# Autodesk Inventor assembly: ASY PNS 1650 filter-distribution-system 1000
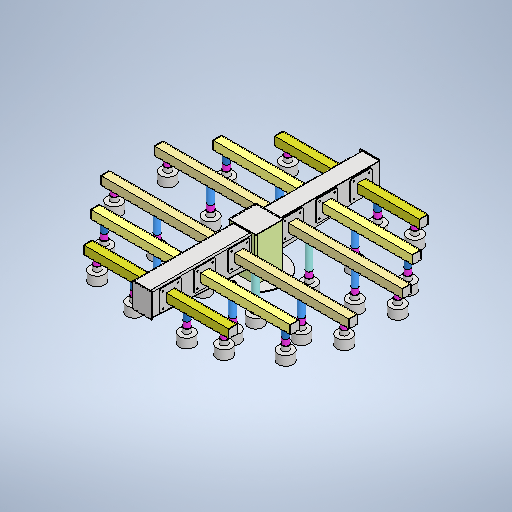
[picture p0: Inventor's stored thumbnail of the model, 512x512]
Saved by Autodesk Inventor 2025.3 (Build 293356030, 356C)
## iProperties
Created: 2025-06-24
Part Number: ASY PNS 1650 filter-distribution-system 1000
Document SubType Name: Assembly
Designer: admin
Author: user
## Documents named in this file (12)
- C:\Users\admin\Yandex.Disk\home pc\Inventor\SLM-Salemal\ASY PNS 1650 filter-distribution-system 1000.iam
- C:\Users\admin\Yandex.Disk\home pc\Inventor\SLM-Salemal\PNS 169859 DIM filter-distribution-system 1000.ipt
- C:\Users\admin\Yandex.Disk\home pc\Inventor\SLM-Salemal\PNS 1651 FDS MAIN  FLANGE.ipt
- C:\Users\admin\Yandex.Disk\home pc\Inventor\SLM-Salemal\PNS 1652 FDS Central tube wall.ipt
- C:\Users\admin\Yandex.Disk\home pc\Inventor\SLM-Salemal\ASY PNS FDS way1_1600.iam
- C:\Users\admin\Yandex.Disk\home pc\Inventor\SLM-Salemal\ASY PNS 1662 FDS way 2.iam
- C:\Users\admin\Yandex.Disk\home pc\Inventor\SLM-Salemal\ASY PNS FDS way3_1600.iam
- C:\Users\admin\Yandex.Disk\home pc\Inventor\SLM-Salemal\PNS 1665 FDS 1000 CUP 1.ipt
- C:\Users\admin\Yandex.Disk\home pc\Inventor\SLM-Salemal\SLM 1422 BOTTOM FDS diameter way up.ipt
- C:\Users\admin\Yandex.Disk\home pc\Inventor\SLM-Salemal\SLM 1423 BOTTOM FDS diameter way down.ipt
- C:\Users\admin\Yandex.Disk\home pc\Inventor\SLM-Salemal\SLM 1424 FDS diam way cup.ipt
- C:\Users\admin\Yandex.Disk\home pc\Inventor\SLM-Salemal\SLM 1421 FDS Diam way flange 1.ipt
## Components (24 placed, 12 different names)
1. PNS 169859 DIM filter-distribution-system 1000.ipt:1 — Mate:5, Mate:4
2. PNS 1651 FDS MAIN  FLANGE.ipt:1 — Flush:1, Mate:5, Flush:5, Flush:6
3. PNS 1652 FDS Central tube wall.ipt:1 — Flush:1, Flush:4, Flush:3, Mate:6, Rigid:1, Flush:6, Rigid:7
4. PNS 1652 FDS Central tube wall.ipt:2 — Rigid:1, Mate:5, Flush:5, Rigid:21
5. ASY PNS FDS way1_1600.iam:1 [sub-assembly] — Rigid:12
6. ASY PNS 1662 FDS way 2.iam:1 [sub-assembly] — Rigid:10
7. ASY PNS FDS way3_1600.iam:1 [sub-assembly] — Rigid:8
8. ASY PNS FDS way1_1600.iam:2 [sub-assembly] — Rigid:16
9. ASY PNS FDS way1_1600.iam:3 [sub-assembly] — Rigid:13
10. ASY PNS 1662 FDS way 2.iam:2 [sub-assembly] — Rigid:11
11. ASY PNS 1662 FDS way 2.iam:3 [sub-assembly] — Rigid:18
12. ASY PNS 1662 FDS way 2.iam:4 [sub-assembly] — Rigid:14
13. ASY PNS FDS way3_1600.iam:2 [sub-assembly] — Rigid:9
14. ASY PNS FDS way3_1600.iam:3 [sub-assembly] — Rigid:15
15. ASY PNS FDS way3_1600.iam:4 [sub-assembly] — Rigid:19
16. PNS 1665 FDS 1000 CUP 1.ipt:1 — Flush:4, Flush:3, Mate:6
17. SLM 1422 BOTTOM FDS diameter way up:1 — Rigid:9, Rigid:11, Rigid:16
18. SLM 1423 BOTTOM FDS diameter way down:1 — Rigid:8, Rigid:10, Rigid:12, Rigid:20, Rigid:21
19. SLM 1424 FDS diam way cup:1
20. ASY PNS FDS way1_1600:4 [sub-assembly] — Rigid:17
21. SLM 1422 BOTTOM FDS diameter way up:2 — Rigid:17, Rigid:18, Rigid:19
22. SLM 1423 BOTTOM FDS diameter way down:2 — Rigid:7, Rigid:13, Rigid:14, Rigid:15
23. SLM 1424 FDS diam way cup:2
24. SLM 1421 FDS Diam way flange 1:1 — Rigid:20
## Relationships (29: WeldJoint 20, Flush 5, Mate 4)
- Mate:5: PNS 169859 DIM filter-distribution-system 1000.ipt:1
- Mate:4: PNS 169859 DIM filter-distribution-system 1000.ipt:1
- Flush:1: PNS 1651 FDS MAIN  FLANGE.ipt:1 ↔ PNS 1652 FDS Central tube wall.ipt:1
- Flush:4: PNS 1652 FDS Central tube wall.ipt:1 ↔ PNS 1665 FDS 1000 CUP 1.ipt:1
- Flush:3: PNS 1652 FDS Central tube wall.ipt:1 ↔ PNS 1665 FDS 1000 CUP 1.ipt:1
- Mate:6: PNS 1652 FDS Central tube wall.ipt:1 ↔ PNS 1665 FDS 1000 CUP 1.ipt:1
- Rigid:1 [WeldJoint]: PNS 1652 FDS Central tube wall.ipt:1 ↔ PNS 1652 FDS Central tube wall.ipt:2
- [WeldJoint]: SLM 1422 BOTTOM FDS diameter way up:1 ↔ SLM 1423 BOTTOM FDS diameter way down:1
- [WeldJoint]: SLM 1423 BOTTOM FDS diameter way down:1 ↔ SLM 1424 FDS diam way cup:1
- Mate:5: PNS 1651 FDS MAIN  FLANGE.ipt:1 ↔ PNS 1652 FDS Central tube wall.ipt:2
- Flush:5: PNS 1651 FDS MAIN  FLANGE.ipt:1 ↔ PNS 1652 FDS Central tube wall.ipt:2
- Flush:6: PNS 1651 FDS MAIN  FLANGE.ipt:1 ↔ PNS 1652 FDS Central tube wall.ipt:1
- [WeldJoint]: SLM 1422 BOTTOM FDS diameter way up:2 ↔ SLM 1423 BOTTOM FDS diameter way down:2
- [WeldJoint]: SLM 1423 BOTTOM FDS diameter way down:2 ↔ SLM 1424 FDS diam way cup:2
- Rigid:7 [WeldJoint]: PNS 1652 FDS Central tube wall.ipt:1 ↔ SLM 1423 BOTTOM FDS diameter way down:2
- Rigid:8 [WeldJoint]: ASY PNS FDS way3_1600.iam:1 ↔ SLM 1423 BOTTOM FDS diameter way down:1
- Rigid:9 [WeldJoint]: ASY PNS FDS way3_1600.iam:2 ↔ SLM 1422 BOTTOM FDS diameter way up:1
- Rigid:10 [WeldJoint]: ASY PNS 1662 FDS way 2.iam:1 ↔ SLM 1423 BOTTOM FDS diameter way down:1
- Rigid:11 [WeldJoint]: ASY PNS 1662 FDS way 2.iam:2 ↔ SLM 1422 BOTTOM FDS diameter way up:1
- Rigid:12 [WeldJoint]: ASY PNS FDS way1_1600.iam:1 ↔ SLM 1423 BOTTOM FDS diameter way down:1
- Rigid:13 [WeldJoint]: ASY PNS FDS way1_1600.iam:3 ↔ SLM 1423 BOTTOM FDS diameter way down:2
- Rigid:14 [WeldJoint]: ASY PNS 1662 FDS way 2.iam:4 ↔ SLM 1423 BOTTOM FDS diameter way down:2
- Rigid:15 [WeldJoint]: ASY PNS FDS way3_1600.iam:3 ↔ SLM 1423 BOTTOM FDS diameter way down:2
- Rigid:16 [WeldJoint]: ASY PNS FDS way1_1600.iam:2 ↔ SLM 1422 BOTTOM FDS diameter way up:1
- Rigid:17 [WeldJoint]: ASY PNS FDS way1_1600:4 ↔ SLM 1422 BOTTOM FDS diameter way up:2
- Rigid:18 [WeldJoint]: ASY PNS 1662 FDS way 2.iam:3 ↔ SLM 1422 BOTTOM FDS diameter way up:2
- Rigid:19 [WeldJoint]: ASY PNS FDS way3_1600.iam:4 ↔ SLM 1422 BOTTOM FDS diameter way up:2
- Rigid:20 [WeldJoint]: SLM 1423 BOTTOM FDS diameter way down:1 ↔ SLM 1421 FDS Diam way flange 1:1
- Rigid:21 [WeldJoint]: PNS 1652 FDS Central tube wall.ipt:2 ↔ SLM 1423 BOTTOM FDS diameter way down:1
## Named parameters: d49_d114 = 0 mm, d50_d115 = 0 mm
